# Autodesk Inventor assembly: Bracket Assembly MK1
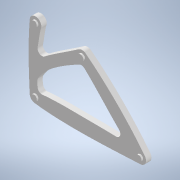
[picture p0: Inventor's stored thumbnail of the model, 180x180]
Saved by Autodesk Inventor 2021 (Build 250183000, 183)
## iProperties
Created: 2021-05-12
Part Number: Bracket Assembly MK1
Document SubType Name: Assembly
Designer: Jawal
Author: Jawal
## Documents named in this file (3)
- C:\Users\Jawal\Documents\UNI\PART III\Semester 1\MECHENG 334\Project B\Concept Design\Bracket Assembly MK1.iam
- C:\Users\Jawal\Documents\UNI\PART III\Semester 1\MECHENG 334\Project B\Concept Design\Bracket Concept MK2.ipt
- C:\Users\Jawal\Documents\UNI\PART III\Semester 1\MECHENG 334\Project B\Concept Design\Pin.ipt
## Components (5 placed, 2 different names)
1. Bracket Concept MK2:1 — Rigid:1, Rigid:2, Rigid:3, Rigid:4
2. Pin:1 — Rigid:1
3. Pin:2 — Rigid:2
4. Pin:3 — Rigid:3
5. Pin:4 — Rigid:4
## Relationships (4: WeldJoint 4)
- Rigid:1 [WeldJoint]: Bracket Concept MK2:1 ↔ Pin:1
- Rigid:2 [WeldJoint]: Bracket Concept MK2:1 ↔ Pin:2
- Rigid:3 [WeldJoint]: Bracket Concept MK2:1 ↔ Pin:3
- Rigid:4 [WeldJoint]: Bracket Concept MK2:1 ↔ Pin:4
